# Autodesk Inventor assembly: AM14U3 Long Frame Half
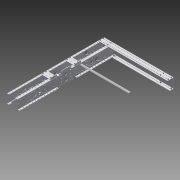
[picture p0: Inventor's stored thumbnail of the model, 180x180]
Saved by Autodesk Inventor 2016 SP1 (Build 200210100, 210)
## iProperties
Created: 2015-12-05
Part Number: AM14U3 Long Frame Half
Document SubType Name: Assembly
Designer: PhillipD
Author: PhillipD
Revision Number: ANY
## Documents named in this file (10)
- D:\FIRST\FRC KOP 2016\FRC KOP 2016\Drive Base\Parts\AM14U3 Long Frame Half.iam
- D:\FIRST\FRC KOP 2016\FRC KOP 2016\Drive Base\Parts\10-32x0500_shcs_HX-SHCS 0.19-32x1.375x1-C.ipt
- D:\FIRST\FRC KOP 2016\FRC KOP 2016\Drive Base\Parts\10-32 Nylock Nut.ipt
- D:\FIRST\FRC KOP 2016\FRC KOP 2016\Drive Base\Parts\Churro 3375.ipt
- D:\FIRST\FRC KOP 2016\FRC KOP 2016\Drive Base\Parts\FHTS 0.25-20-0.75_FHTS 0.25-20-G-0.75-C.ipt
- D:\FIRST\FRC KOP 2016\FRC KOP 2016\Drive Base\Parts\AM14U3 End Sheet Long.ipt
- D:\FIRST\FRC KOP 2016\FRC KOP 2016\Drive Base\Parts\AM14U3 Inside Sheet Rev2.ipt
- D:\FIRST\FRC KOP 2016\FRC KOP 2016\Drive Base\Parts\AM14U3 Outside Sheet Rev1_DefaultSM-FLAT-PATTERN.ipt
- D:\FIRST\FRC KOP 2016\FRC KOP 2016\Drive Base\Parts\am-2954 AM14U2 2x3 Hole Bracket.ipt
- D:\FIRST\FRC KOP 2016\FRC KOP 2016\Drive Base\Parts\Churro 16250.ipt
## Components (60 placed, 60 different names)
1. 10-32x0500_shcs_HX-SHCS 0.19-32x1.375x1-C_80
2. 10-32x0500_shcs_HX-SHCS 0.19-32x1.375x1-C_81
3. 10-32x0500_shcs_HX-SHCS 0.19-32x1.375x1-C_82
4. 10-32x0500_shcs_HX-SHCS 0.19-32x1.375x1-C_83
5. 10-32x0500_shcs_HX-SHCS 0.19-32x1.375x1-C_84
6. 10-32x0500_shcs_HX-SHCS 0.19-32x1.375x1-C_85
7. 10-32 Nylock Nut_86
8. 10-32 Nylock Nut_87
9. 10-32 Nylock Nut_88
10. 10-32 Nylock Nut_89
11. 10-32 Nylock Nut_90
12. 10-32 Nylock Nut_91
13. 10-32x0500_shcs_HX-SHCS 0.19-32x1.375x1-C_92
14. 10-32x0500_shcs_HX-SHCS 0.19-32x1.375x1-C_93
15. 10-32x0500_shcs_HX-SHCS 0.19-32x1.375x1-C_94
16. 10-32x0500_shcs_HX-SHCS 0.19-32x1.375x1-C_95
17. 10-32x0500_shcs_HX-SHCS 0.19-32x1.375x1-C_96
18. 10-32x0500_shcs_HX-SHCS 0.19-32x1.375x1-C_97
19. 10-32 Nylock Nut_98
20. 10-32 Nylock Nut_99
21. 10-32 Nylock Nut_100
22. 10-32 Nylock Nut_101
23. 10-32 Nylock Nut_102
24. 10-32 Nylock Nut_103
25. 10-32x0500_shcs_HX-SHCS 0.19-32x1.375x1-C_104
26. 10-32x0500_shcs_HX-SHCS 0.19-32x1.375x1-C_105
27. 10-32x0500_shcs_HX-SHCS 0.19-32x1.375x1-C_106
28. 10-32x0500_shcs_HX-SHCS 0.19-32x1.375x1-C_107
29. 10-32x0500_shcs_HX-SHCS 0.19-32x1.375x1-C_108
30. 10-32x0500_shcs_HX-SHCS 0.19-32x1.375x1-C_109
31. 10-32x0500_shcs_HX-SHCS 0.19-32x1.375x1-C_110
32. 10-32x0500_shcs_HX-SHCS 0.19-32x1.375x1-C_111
33. 10-32 Nylock Nut_112
34. 10-32 Nylock Nut_113
35. 10-32 Nylock Nut_114
36. 10-32 Nylock Nut_115
37. 10-32 Nylock Nut_116
38. 10-32 Nylock Nut_117
39. 10-32 Nylock Nut_118
40. 10-32 Nylock Nut_119
41. Churro 3375_120
42. Churro 3375_121
43. Churro 3375_122
44. Churro 3375_123
45. FHTS 0.25-20-0.75_FHTS 0.25-20-G-0.75-C_125
46. FHTS 0.25-20-0.75_FHTS 0.25-20-G-0.75-C_126
47. FHTS 0.25-20-0.75_FHTS 0.25-20-G-0.75-C_127
48. FHTS 0.25-20-0.75_FHTS 0.25-20-G-0.75-C_128
49. FHTS 0.25-20-0.75_FHTS 0.25-20-G-0.75-C_129
50. FHTS 0.25-20-0.75_FHTS 0.25-20-G-0.75-C_130
51. FHTS 0.25-20-0.75_FHTS 0.25-20-G-0.75-C_131
52. FHTS 0.25-20-0.75_FHTS 0.25-20-G-0.75-C_132
53. FHTS 0.25-20-0.75_FHTS 0.25-20-G-0.75-C_133
54. FHTS 0.25-20-0.75_FHTS 0.25-20-G-0.75-C_134 — Mate:1, Mate:2
55. AM14U3 End Sheet Long_135
56. AM14U3 Inside Sheet Rev2_136 — Insert:1
57. AM14U3 Outside Sheet Rev1_DefaultSM-FLAT-PATTERN_137
58. am-2954 AM14U2 2x3 Hole Bracket_138
59. am-2954 AM14U2 2x3 Hole Bracket_139
60. Churro 16250:1 — Insert:1, Mate:1, Mate:2
## Relationships (3: Mate 2, Insert 1)
- Insert:1: AM14U3 Inside Sheet Rev2_136 ↔ Churro 16250:1
- Mate:1: FHTS 0.25-20-0.75_FHTS 0.25-20-G-0.75-C_134 ↔ Churro 16250:1
- Mate:2 (3.175 mm): FHTS 0.25-20-0.75_FHTS 0.25-20-G-0.75-C_134 ↔ Churro 16250:1
